# Autodesk Inventor assembly: Gripper_re
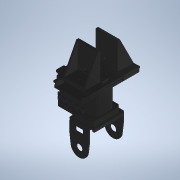
[picture p0: Inventor's stored thumbnail of the model, 180x180]
Saved by Autodesk Inventor 2021.3 (Build 253353000, 353)
## iProperties
Created: 2022-02-03
Part Number: Gripper_re
Document SubType Name: Assembly
Designer: epm01
Author: epm01
## Documents named in this file (3)
- D:\Archivos\2020-2\Papime\Banco_serial\Gripper_re.iam
- D:\Archivos\2020-2\Papime\Banco_serial\Robot_gripper\phantomx-pincher-robot-arm-kit-mark-ii-1.snapshot.1\GripperBody v4.ipt
- D:\Archivos\2020-2\Papime\Banco_serial\Robot_gripper\phantomx-pincher-robot-arm-kit-mark-ii-1.snapshot.1\LeftFinger v2.ipt
## Components (3 placed, 2 different names)
1. GripperBody v4:1 — Coincidencia:1, Coincidencia:2, Coincidencia:3, Coincidencia:4
2. LeftFinger v2:1 — Coincidencia:1, Coincidencia:2
3. LeftFinger v2:2 — Coincidencia:3, Coincidencia:4
## Relationships (4: Mate 4)
- Coincidencia:1 [Mate]: GripperBody v4:1 ↔ LeftFinger v2:1
- Coincidencia:2 [Mate]: GripperBody v4:1 ↔ LeftFinger v2:1
- Coincidencia:3 [Mate]: GripperBody v4:1 ↔ LeftFinger v2:2
- Coincidencia:4 [Mate]: GripperBody v4:1 ↔ LeftFinger v2:2
